# Autodesk Inventor assembly: model
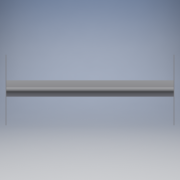
[picture p0: Inventor's stored thumbnail of the model, 180x180]
Saved by Autodesk Inventor 2018.2 (Build 222227000, 227)
## iProperties
Created: 2018-02-25
Part Number: model
Material: 一般
Document SubType Name: Assembly
Designer: ku_sk
Author: ku_sk
## Documents named in this file (3)
- C:\Users\ku_sk\Documents\Inventor\AeroCAD2018\設計\Rr.wing\model.iam
- C:\Users\ku_sk\Documents\Inventor\AeroCAD2018\設計\Rr.wing\parts\frap.ipt
- C:\Users\ku_sk\Documents\Inventor\AeroCAD2018\設計\Rr.wing\parts\endplate.ipt
## Components (3 placed, 2 different names)
1. frap:1 — フラッシュ:1, メイト:1, メイト:2, 角度:2, メイト:3, メイト:4
2. endplate:1 — メイト:1, フラッシュ:2
3. endplate:2 — メイト:2, 角度:1, フラッシュ:2, メイト:4
## Relationships (8: Mate 4, Flush 2, Angle 2)
- フラッシュ:1 [Flush]: frap:1
- メイト:1 [Mate]: frap:1 ↔ endplate:1
- メイト:2 [Mate]: frap:1 ↔ endplate:2
- 角度:1 [Angle] (0 deg): endplate:2
- フラッシュ:2 [Flush]: endplate:1 ↔ endplate:2
- 角度:2 [Angle] (-10 deg): frap:1
- メイト:3 [Mate]: frap:1
- メイト:4 [Mate]: frap:1 ↔ endplate:2
